# Autodesk Inventor assembly: Body
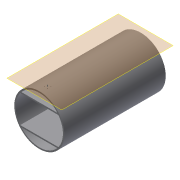
[picture p0: Inventor's stored thumbnail of the model, 180x180]
Saved by Autodesk Inventor 2017 (Build 210142000, 142)
## iProperties
Created: 2017-03-13
Part Number: Body
Document SubType Name: Assembly
Designer: zallen
Author: zallen
## Documents named in this file (4)
- C:\Users\zallen\Documents\Autodesk Inventor Projects\LaundryRobot_v0.1\Body.iam
- C:\Users\zallen\Documents\Autodesk Inventor Projects\LaundryRobot_v0.1\Chassis.ipt
- C:\Users\zallen\Documents\Autodesk Inventor Projects\Stepper Motor\Двигатель.ipt
- C:\Users\zallen\Documents\Inventor\Content Center Files\R2017\en-US\ISO 7047 (H)\ISO 7047 - M3.5x5 - 4.8 - H.ipt
## Components (3 placed, 3 different names)
1. Stepper Motor:1 — Mate:1
2. Chassis:1 — Angle:1, Tangent:1, Flush:1
3. ISO 7047 (H) M3.5x5 - 4.8 - H:1 — Mate:1
## Relationships (4: Angle 1, Tangent 1, Flush 1, Mate 1)
- Angle:1 (0 deg): Chassis:1
- Tangent:1: Chassis:1
- Flush:1: Chassis:1
- Mate:1: Stepper Motor:1 ↔ ISO 7047 (H) M3.5x5 - 4.8 - H:1
